# Autodesk Inventor assembly: SyncHub_Assembly
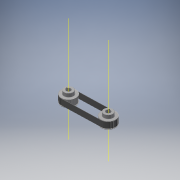
[picture p0: Inventor's stored thumbnail of the model, 180x180]
Saved by Autodesk Inventor 2018 (Build 220112000, 112)
## iProperties
Created: 2018-05-08
Part Number: SyncHub_Assembly
Document SubType Name: Assembly
Designer: P136265
Author: P136265
## Documents named in this file (3)
- C:\Users\P136265\Documents\GitHub\mecanum-cad\SyncHub_Assembly.iam
- C:\Users\P136265\Documents\GitHub\mecanum-cad\Synchronous Belt1.ipt
- C:\Users\P136265\Documents\GitHub\mecanum-cad\Synchronous Pulley21.ipt
## Components (3 placed, 2 different names)
1. Synchronous Belt:1 — Mate:2, Flush:2, Mate:3
2. Synchronous Pulley2:1 — Mate:2, Flush:2, Flush:3
3. Synchronous Pulley2:2 — Mate:3, Flush:3
## Relationships (4: Mate 2, Flush 2)
- Mate:2: Synchronous Belt:1 ↔ Synchronous Pulley2:1
- Flush:2 (-2 mm): Synchronous Belt:1 ↔ Synchronous Pulley2:1
- Mate:3: Synchronous Belt:1 ↔ Synchronous Pulley2:2
- Flush:3: Synchronous Pulley2:1 ↔ Synchronous Pulley2:2
